# Autodesk Inventor assembly: PrinterAssambly
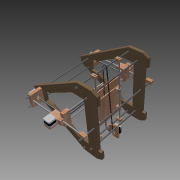
[picture p0: Inventor's stored thumbnail of the model, 180x180]
Saved by Autodesk Inventor 2014 (Build 180170000, 170)
## iProperties
Created: 2013-12-10
Part Number: PrinterAssambly
Document SubType Name: Assembly
Designer: Bram
Author: Bram
## Documents named in this file (28)
- D:\gDrive\Google Drive\Hobby\3D Printer\3D printer\Inventor\PrinterAssambly.iam
- D:\gDrive\Google Drive\Hobby\3D Printer\3D printer\Inventor\A_Frame_V2.ipt
- D:\gDrive\Google Drive\Hobby\3D Printer\3D printer\Inventor\Rods\370_Thread.ipt
- D:\gDrive\Google Drive\Hobby\3D Printer\3D printer\Inventor\Rods\508_Thread.ipt
- D:\gDrive\Google Drive\Hobby\3D Printer\3D printer\Inventor\Z_MotorMount_RodHolder__Part1_V2.ipt
- D:\gDrive\Google Drive\Hobby\3D Printer\3D printer\Inventor\Rods\354_Side_Up.ipt
- D:\gDrive\Google Drive\Hobby\3D Printer\3D printer\Inventor\Z_MotorMount_RodHolder_Part2_V2.ipt
- D:\gDrive\Google Drive\Hobby\3D Printer\3D printer\Inventor\NEMA17.ipt
- D:\gDrive\Google Drive\Hobby\3D Printer\3D printer\Inventor\Rods\210_Thread.ipt
- D:\gDrive\Google Drive\Hobby\3D Printer\3D printer\Inventor\Top_RodHolder.ipt
- D:\gDrive\Google Drive\Hobby\3D Printer\3D printer\Inventor\Rods\457.ipt
- D:\gDrive\Google Drive\Hobby\3D Printer\3D printer\Inventor\X_Top_MotorSide_V3.ipt
- D:\gDrive\Google Drive\Hobby\3D Printer\3D printer\Inventor\LM8UU.ipt
- D:\gDrive\Google Drive\Hobby\3D Printer\3D printer\Inventor\X_Top_PullySide_V2.ipt
- D:\gDrive\Google Drive\Hobby\3D Printer\3D printer\Inventor\X_Bottem_MotorSide_V3.ipt
- D:\gDrive\Google Drive\Hobby\3D Printer\3D printer\Inventor\PrinterAssambly\Design Accelerator\Synchronous Belts Transmission1.iam
- D:\gDrive\Google Drive\Hobby\3D Printer\3D printer\Inventor\Y_MotorMount.ipt
- D:\gDrive\Google Drive\Hobby\3D Printer\3D printer\Inventor\608ZZBearing.ipt
- D:\gDrive\Google Drive\Hobby\3D Printer\3D printer\Inventor\Timping Pully.ipt
- D:\gDrive\Google Drive\Hobby\3D Printer\3D printer\Inventor\X_Carriage_WithBearings.ipt
- D:\gDrive\Google Drive\Hobby\3D Printer\3D printer\Inventor\Rods\406.ipt
- D:\gDrive\Google Drive\Hobby\3D Printer\3D printer\Inventor\Y_RodClam_Bed.ipt
- D:\gDrive\Google Drive\Hobby\3D Printer\3D printer\Inventor\Print_BottemPlate.ipt
- D:\gDrive\Google Drive\Hobby\3D Printer\3D printer\Inventor\Print_TopPlate.ipt
- D:\gDrive\Google Drive\Hobby\3D Printer\3D printer\Inventor\Heatbed_Standoff.ipt
- D:\gDrive\Google Drive\Hobby\3D Printer\3D printer\Inventor\Heatbed.ipt
- D:\gDrive\Google Drive\Hobby\3D Printer\3D printer\Inventor\PrinterAssambly\Design Accelerator\Synchronous Belts Transmission2.iam
- D:\gDrive\Google Drive\Hobby\3D Printer\3D printer\Inventor\BarClamp_V3.ipt
## Components (59 placed, 26 different names)
1. A_Frame_V2:1 — Mate:8, Mate:37
2. A_Frame_V2:2 — Mate:4, Flush:4, Mate:5, Flush:5, Mate:6, Flush:6, Mate:7, Flush:7, Mate:9, Mate:10, Mate:14, Mate:17
3. 370_Thread:3 — Mate:4, Flush:4, Mate:8, Mate:88, Mate:91, Mate:141, Mate:143
4. 370_Thread:4 — Mate:5, Flush:5, Mate:87
5. 370_Thread:5 — Mate:7, Flush:7
6. 370_Thread:6 — Mate:6, Flush:6, Mate:92, Mate:137, Mate:139
7. 508_Thread:1 — Mate:9, Mate:15, Mate:19, Mate:36
8. 508_Thread:2 — Mate:10, Mate:16, Mate:20, Mate:35, Mate:39
9. 508_Thread:3 — Mate:14, Mate:26, Mate:46
10. Z_MotorMount_RodHolder__Part1_V2:1 — Mate:15, Mate:16, Mate:17, Mate:18, Mate:21, Mate:22
11. 354_Side_Up:1 — Mate:18, Mate:25, Mate:62, Mate:69
12. Z_MotorMount_RodHolder_Part2_V2:1 — Mate:19, Mate:20, Mate:21
13. NEMA17:1 — Mate:22, Mate:23, Mate:24
14. 210_Thread:1 — Mate:23, Mate:24, Mate:63, Mate:68
15. Top_RodHolder:1 — Mate:25, Mate:26
16. Z_MotorMount_RodHolder__Part1_V2:2 — Mate:35, Mate:36, Mate:37, Mate:38, Mate:40, Mate:41, Mate:42
17. 354_Side_Up:2 — Mate:38, Mate:45, Mate:66, Mate:72
18. Z_MotorMount_RodHolder_Part2_V2:2 — Mate:39, Mate:40
19. NEMA17:3 — Mate:41, Mate:42, Mate:43, Mate:44
20. 210_Thread:2 — Mate:43, Mate:44, Mate:67, Mate:71
21. Top_RodHolder:2 — Mate:45, Mate:46
22. X_Top_MotorSide_V3:1 — Mate:58, Mate:59, Mate:60, Mate:61, Mate:63, Mate:70
23. LM8UU:1 — Mate:58, Mate:59, Mate:62
24. NEMA17:4 — Mate:60, Mate:61, Mate:83, Mate:84
25. X_Top_PullySide_V2:1 — Mate:65, Flush:10, Mate:67, Mate:73, Mate:82
26. LM8UU:2 — Mate:65, Flush:10, Mate:66
27. X_Bottem_MotorSide_V3:1 — Mate:68, Mate:69, Mate:70, Mate:75, Mate:76
28. X_Bottem_MotorSide_V3:2 — Mate:71, Mate:72, Mate:73, Mate:74, Flush:11, Mate:77, Flush:12
29. 457:1 — Mate:74, Mate:75, Flush:11, Mate:97
30. 457:2 — Mate:76, Mate:77, Flush:12, Mate:98
31. Synchronous Belts Transmission:1 [sub-assembly] — Mate:82, Mate:83, Mate:84
32. Y_MotorMount:1 — Mate:87, Mate:88, Mate:89, Mate:90, Flush:13
33. NEMA17:5 — Mate:89, Mate:90, Mate:95
34. 608ZZBearing:1 — Mate:91, Mate:93, Mate:96, Flush:21
35. 608ZZBearing:2 — Mate:92, Mate:93
36. Timping Pully:1 — Mate:95, Mate:96, Flush:13
37. X_Carriage_WithBearings:1 — Mate:97, Mate:98
38. 406:1 — Mate:108, Mate:109, Mate:140, Mate:142, Flush:22
39. 406:2 — Mate:110, Mate:111, Mate:138, Mate:144
40. LM8UU:3 — Mate:108, Mate:112, Mate:113
41. LM8UU:4 — Mate:110, Mate:116, Flush:18
42. LM8UU:5 — Mate:109, Mate:114, Flush:16
43. LM8UU:6 — Mate:111, Mate:115, Flush:17
44. Y_RodClam_Bed:1 — Mate:116, Flush:18, Mate:117, Mate:118, Mate:122, Mate:123
45. Y_RodClam_Bed:3 — Mate:112, Mate:113, Mate:119, Mate:120, Flush:19
46. Y_RodClam_Bed:4 — Mate:114, Flush:16, Mate:119, Mate:120, Mate:121
47. Y_RodClam_Bed:5 — Mate:115, Flush:17, Mate:117, Mate:118, Mate:121
48. Print_BottemPlate:1 — Mate:122, Mate:123, Flush:19, Mate:124, Mate:125, Flush:20
49. Print_TopPlate:1 — Mate:124, Mate:125, Flush:20, Mate:126, Mate:127, Mate:128, Mate:129, Mate:130, Mate:131, Mate:132, Mate:133
50. Heatbed_Standoff:1 — Mate:126, Mate:127, Mate:136
51. Heatbed_Standoff:2 — Mate:128, Mate:129
52. Heatbed_Standoff:3 — Mate:130, Mate:131, Mate:134, Mate:135
53. Heatbed_Standoff:4 — Mate:132, Mate:133
54. Heatbed:1 — Mate:134, Mate:135, Mate:136
55. Synchronous Belts Transmission:2 [sub-assembly] — Flush:21
56. BarClamp_V3:1 — Mate:137, Mate:138
57. BarClamp_V3:2 — Mate:139, Mate:140
58. BarClamp_V3:3 — Mate:141, Mate:142, Flush:22
59. BarClamp_V3:4 — Mate:143, Mate:144
## Relationships (117: Mate 102, Flush 15)
- Mate:4: A_Frame_V2:2 ↔ 370_Thread:3
- Flush:4 (-10 mm): A_Frame_V2:2 ↔ 370_Thread:3
- Mate:5: A_Frame_V2:2 ↔ 370_Thread:4
- Flush:5 (10 mm): A_Frame_V2:2 ↔ 370_Thread:4
- Mate:6: A_Frame_V2:2 ↔ 370_Thread:6
- Flush:6 (10 mm): A_Frame_V2:2 ↔ 370_Thread:6
- Mate:7: A_Frame_V2:2 ↔ 370_Thread:5
- Flush:7 (10 mm): A_Frame_V2:2 ↔ 370_Thread:5
- Mate:8: A_Frame_V2:1 ↔ 370_Thread:3
- Mate:9: A_Frame_V2:2 ↔ 508_Thread:1
- Mate:10: A_Frame_V2:2 ↔ 508_Thread:2
- Mate:14: A_Frame_V2:2 ↔ 508_Thread:3
- Mate:15: 508_Thread:1 ↔ Z_MotorMount_RodHolder__Part1_V2:1
- Mate:16: 508_Thread:2 ↔ Z_MotorMount_RodHolder__Part1_V2:1
- Mate:17: A_Frame_V2:2 ↔ Z_MotorMount_RodHolder__Part1_V2:1
- Mate:18: Z_MotorMount_RodHolder__Part1_V2:1 ↔ 354_Side_Up:1
- Mate:19: 508_Thread:1 ↔ Z_MotorMount_RodHolder_Part2_V2:1
- Mate:20: 508_Thread:2 ↔ Z_MotorMount_RodHolder_Part2_V2:1
- Mate:21 (1 mm): Z_MotorMount_RodHolder__Part1_V2:1 ↔ Z_MotorMount_RodHolder_Part2_V2:1
- Mate:22: Z_MotorMount_RodHolder__Part1_V2:1 ↔ NEMA17:1
- Mate:23: NEMA17:1 ↔ 210_Thread:1
- Mate:24: NEMA17:1 ↔ 210_Thread:1
- Mate:25: 354_Side_Up:1 ↔ Top_RodHolder:1
- Mate:26: 508_Thread:3 ↔ Top_RodHolder:1
- Mate:35: 508_Thread:2 ↔ Z_MotorMount_RodHolder__Part1_V2:2
- Mate:36: 508_Thread:1 ↔ Z_MotorMount_RodHolder__Part1_V2:2
- Mate:37: A_Frame_V2:1 ↔ Z_MotorMount_RodHolder__Part1_V2:2
- Mate:38: Z_MotorMount_RodHolder__Part1_V2:2 ↔ 354_Side_Up:2
- Mate:39: 508_Thread:2 ↔ Z_MotorMount_RodHolder_Part2_V2:2
- Mate:40 (1 mm): Z_MotorMount_RodHolder__Part1_V2:2 ↔ Z_MotorMount_RodHolder_Part2_V2:2
- Mate:41: Z_MotorMount_RodHolder__Part1_V2:2 ↔ NEMA17:3
- Mate:42: Z_MotorMount_RodHolder__Part1_V2:2 ↔ NEMA17:3
- Mate:43: NEMA17:3 ↔ 210_Thread:2
- Mate:44: NEMA17:3 ↔ 210_Thread:2
- Mate:45: 354_Side_Up:2 ↔ Top_RodHolder:2
- Mate:46: 508_Thread:3 ↔ Top_RodHolder:2
- Mate:58: X_Top_MotorSide_V3:1 ↔ LM8UU:1
- Mate:59 (-2 mm): X_Top_MotorSide_V3:1 ↔ LM8UU:1
- Mate:60: X_Top_MotorSide_V3:1 ↔ NEMA17:4
- Mate:61: X_Top_MotorSide_V3:1 ↔ NEMA17:4
- Mate:62: 354_Side_Up:1 ↔ LM8UU:1
- Mate:63: 210_Thread:1 ↔ X_Top_MotorSide_V3:1
- Mate:65: X_Top_PullySide_V2:1 ↔ LM8UU:2
- Flush:10 (1 mm): X_Top_PullySide_V2:1 ↔ LM8UU:2
- Mate:66: 354_Side_Up:2 ↔ LM8UU:2
- Mate:67: 210_Thread:2 ↔ X_Top_PullySide_V2:1
- Mate:68: 210_Thread:1 ↔ X_Bottem_MotorSide_V3:1
- Mate:69: 354_Side_Up:1 ↔ X_Bottem_MotorSide_V3:1
- Mate:70: X_Top_MotorSide_V3:1 ↔ X_Bottem_MotorSide_V3:1
- Mate:71: 210_Thread:2 ↔ X_Bottem_MotorSide_V3:2
- Mate:72: 354_Side_Up:2 ↔ X_Bottem_MotorSide_V3:2
- Mate:73: X_Top_PullySide_V2:1 ↔ X_Bottem_MotorSide_V3:2
- Mate:74: X_Bottem_MotorSide_V3:2 ↔ 457:1
- Mate:75: X_Bottem_MotorSide_V3:1 ↔ 457:1
- Flush:11: X_Bottem_MotorSide_V3:2 ↔ 457:1
- Mate:76: X_Bottem_MotorSide_V3:1 ↔ 457:2
- Mate:77: X_Bottem_MotorSide_V3:2 ↔ 457:2
- Flush:12: X_Bottem_MotorSide_V3:2 ↔ 457:2
- Mate:82: X_Top_PullySide_V2:1 ↔ Synchronous Belts Transmission:1
- Mate:83: NEMA17:4 ↔ Synchronous Belts Transmission:1
- Mate:84 (1 mm): NEMA17:4 ↔ Synchronous Belts Transmission:1
- Mate:87: 370_Thread:4 ↔ Y_MotorMount:1
- Mate:88: 370_Thread:3 ↔ Y_MotorMount:1
- Mate:89: Y_MotorMount:1 ↔ NEMA17:5
- Mate:90: Y_MotorMount:1 ↔ NEMA17:5
- Mate:91: 370_Thread:3 ↔ 608ZZBearing:1
- Mate:92: 370_Thread:6 ↔ 608ZZBearing:2
- Mate:93: 608ZZBearing:1 ↔ 608ZZBearing:2
- Mate:95: NEMA17:5 ↔ Timping Pully:1
- Mate:96 (1.5 mm): 608ZZBearing:1 ↔ Timping Pully:1
- Flush:13 (-11.8872 mm): Y_MotorMount:1 ↔ Timping Pully:1
- Mate:97: 457:1 ↔ X_Carriage_WithBearings:1
- Mate:98: 457:2 ↔ X_Carriage_WithBearings:1
- Mate:108: 406:1 ↔ LM8UU:3
- Mate:109: 406:1 ↔ LM8UU:5
- Mate:110: 406:2 ↔ LM8UU:4
- Mate:111: 406:2 ↔ LM8UU:6
- Mate:112: LM8UU:3 ↔ Y_RodClam_Bed:3
- Mate:113: LM8UU:3 ↔ Y_RodClam_Bed:3
- Mate:114: LM8UU:5 ↔ Y_RodClam_Bed:4
- Flush:16: LM8UU:5 ↔ Y_RodClam_Bed:4
- Mate:115: LM8UU:6 ↔ Y_RodClam_Bed:5
- Flush:17: LM8UU:6 ↔ Y_RodClam_Bed:5
- Mate:116: LM8UU:4 ↔ Y_RodClam_Bed:1
- Flush:18: LM8UU:4 ↔ Y_RodClam_Bed:1
- Mate:117 (90 mm): Y_RodClam_Bed:1 ↔ Y_RodClam_Bed:5
- Mate:118: Y_RodClam_Bed:1 ↔ Y_RodClam_Bed:5
- Mate:119 (90 mm): Y_RodClam_Bed:3 ↔ Y_RodClam_Bed:4
- Mate:120 (120 mm): Y_RodClam_Bed:3 ↔ Y_RodClam_Bed:4
- Mate:121: Y_RodClam_Bed:4 ↔ Y_RodClam_Bed:5
- Mate:122: Y_RodClam_Bed:1 ↔ Print_BottemPlate:1
- Mate:123 (-140 mm): Y_RodClam_Bed:1 ↔ Print_BottemPlate:1
- Flush:19 (-20 mm): Y_RodClam_Bed:3 ↔ Print_BottemPlate:1
- Mate:124 (4 mm): Print_BottemPlate:1 ↔ Print_TopPlate:1
- Mate:125 (-182.5 mm): Print_BottemPlate:1 ↔ Print_TopPlate:1
- Flush:20: Print_BottemPlate:1 ↔ Print_TopPlate:1
- Mate:126: Print_TopPlate:1 ↔ Heatbed_Standoff:1
- Mate:127: Print_TopPlate:1 ↔ Heatbed_Standoff:1
- Mate:128: Print_TopPlate:1 ↔ Heatbed_Standoff:2
- Mate:129: Print_TopPlate:1 ↔ Heatbed_Standoff:2
- Mate:130: Print_TopPlate:1 ↔ Heatbed_Standoff:3
- Mate:131: Print_TopPlate:1 ↔ Heatbed_Standoff:3
- Mate:132: Print_TopPlate:1 ↔ Heatbed_Standoff:4
- Mate:133: Print_TopPlate:1 ↔ Heatbed_Standoff:4
- Mate:134: Heatbed_Standoff:3 ↔ Heatbed:1
- Mate:135: Heatbed_Standoff:3 ↔ Heatbed:1
- Mate:136: Heatbed_Standoff:1 ↔ Heatbed:1
- Flush:21: 608ZZBearing:1 ↔ Synchronous Belts Transmission:2
- Mate:137: 370_Thread:6 ↔ BarClamp_V3:1
- Mate:138: 406:2 ↔ BarClamp_V3:1
- Mate:139: 370_Thread:6 ↔ BarClamp_V3:2
- Mate:140: 406:1 ↔ BarClamp_V3:2
- Mate:141: 370_Thread:3 ↔ BarClamp_V3:3
- Mate:142: 406:1 ↔ BarClamp_V3:3
- Flush:22 (-10.0076 mm): 406:1 ↔ BarClamp_V3:3
- Mate:143: 370_Thread:3 ↔ BarClamp_V3:4
- Mate:144: 406:2 ↔ BarClamp_V3:4
